# Autodesk Inventor assembly: Moving platform and legs
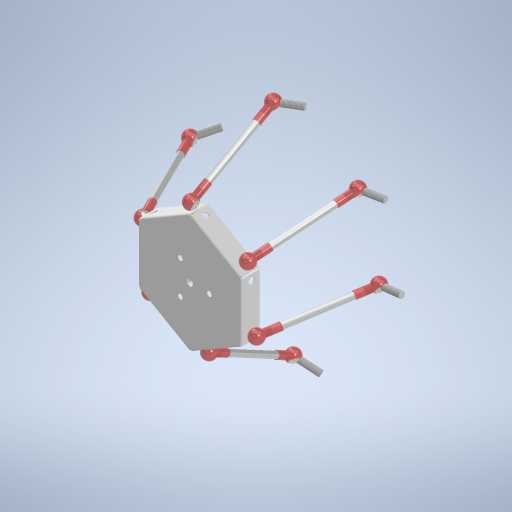
[picture p0: Inventor's stored thumbnail of the model, 512x512]
Saved by Autodesk Inventor 2023 (Build 270158000, 158)
## iProperties
Created: 2022-06-29
Part Number: Moving platform and legs
Document SubType Name: Assembly
Designer: earls
Author: earls
## Documents named in this file (4)
- F:\Documents\Mechatronic Engineering 5.1\Project\CAD\Moving platform and legs.iam
- F:\Documents\Mechatronic Engineering 5.1\Project\CAD\Spherical joint\Assembly1.iam
- F:\Documents\Mechatronic Engineering 5.1\Project\CAD\Moving platform.ipt
- F:\Documents\Mechatronic Engineering 5.1\Project\CAD\Rod qty-6.ipt
## Components (19 placed, 3 different names)
1. Moving platform:1 — Insert:1, Insert:2, Insert:3, Insert:4, Insert:5, Insert:6
2. Assembly1:1 [sub-assembly] — Insert:2, Mate:9, Mate:10
3. Assembly1:2 [sub-assembly] — Insert:6, Mate:5, Mate:6
4. Assembly1:3 [sub-assembly] — Insert:4, Mate:1, Mate:2
5. Assembly1:4 [sub-assembly] — Insert:5, Mate:3, Mate:4
6. Assembly1:5 [sub-assembly] — Insert:3, Mate:11, Mate:12
7. Assembly1:6 [sub-assembly] — Insert:1, Mate:7, Mate:8
8. Rod qty-6:1 — Mate:11, Mate:12, Rotational:3
9. Rod qty-6:2 — Mate:9, Mate:10, Rotational:6
10. Rod qty-6:3 — Mate:7, Mate:8, Rotational:7
11. Rod qty-6:4 — Mate:5, Mate:6, Rotational:2
12. Rod qty-6:5 — Mate:3, Mate:4, Rotational:4
13. Rod qty-6:6 — Mate:1, Mate:2, Rotational:5
14. Assembly1:8 [sub-assembly] — Rotational:3
15. Assembly1:9 [sub-assembly] — Rotational:2
16. Assembly1:11 [sub-assembly] — Rotational:4
17. Assembly1:12 [sub-assembly] — Rotational:7
18. Assembly1:13 [sub-assembly] — Rotational:5
19. Assembly1:14 [sub-assembly] — Rotational:6
## Relationships (24: Mate 12, Insert 6, RevoluteJoint 6)
- Insert:1: Moving platform:1 ↔ Assembly1:6
- Insert:2: Moving platform:1 ↔ Assembly1:1
- Insert:3: Moving platform:1 ↔ Assembly1:5
- Insert:4: Moving platform:1 ↔ Assembly1:3
- Insert:5: Moving platform:1 ↔ Assembly1:4
- Insert:6: Moving platform:1 ↔ Assembly1:2
- Mate:1: Assembly1:3 ↔ Rod qty-6:6
- Mate:2: Assembly1:3 ↔ Rod qty-6:6
- Mate:3: Assembly1:4 ↔ Rod qty-6:5
- Mate:4: Assembly1:4 ↔ Rod qty-6:5
- Mate:5: Assembly1:2 ↔ Rod qty-6:4
- Mate:6: Assembly1:2 ↔ Rod qty-6:4
- Mate:7: Assembly1:6 ↔ Rod qty-6:3
- Mate:8: Assembly1:6 ↔ Rod qty-6:3
- Mate:9: Assembly1:1 ↔ Rod qty-6:2
- Mate:10: Assembly1:1 ↔ Rod qty-6:2
- Mate:11: Assembly1:5 ↔ Rod qty-6:1
- Mate:12: Assembly1:5 ↔ Rod qty-6:1
- Rotational:2 [RevoluteJoint]: Rod qty-6:4 ↔ Assembly1:9
- Rotational:3 [RevoluteJoint]: Rod qty-6:1 ↔ Assembly1:8
- Rotational:4 [RevoluteJoint]: Rod qty-6:5 ↔ Assembly1:11
- Rotational:5 [RevoluteJoint]: Rod qty-6:6 ↔ Assembly1:13
- Rotational:6 [RevoluteJoint]: Rod qty-6:2 ↔ Assembly1:14
- Rotational:7 [RevoluteJoint]: Rod qty-6:3 ↔ Assembly1:12
